# Autodesk Inventor assembly: стенка
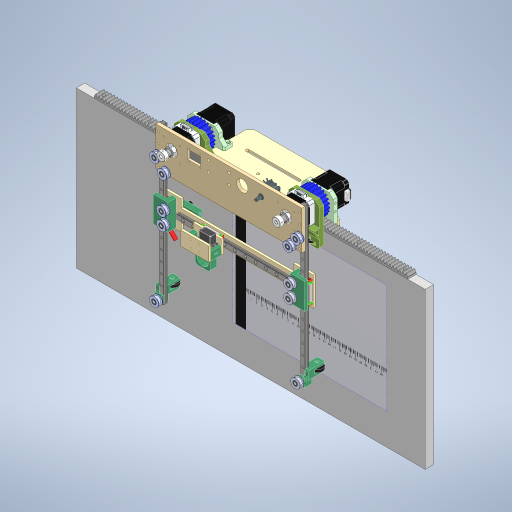
[picture p0: Inventor's stored thumbnail of the model, 512x512]
Saved by Autodesk Inventor 2023.1 (Build 271208000, 208)
## iProperties
Created: 2025-12-01
Part Number: стенка
Document SubType Name: Assembly
Designer: DELL
Author: DELL
## Documents named in this file (9)
- C:\Users\DELL\reposGitHub\VSOSH25-26\models\poligon\poligon.iam
- C:\Users\DELL\reposGitHub\VSOSH25-26\models\plotter\стенка.ipt
- C:\Users\DELL\reposGitHub\VSOSH25-26\models\import\m2_20.ipt
- C:\Users\DELL\reposGitHub\VSOSH25-26\models\actuator\actuator.iam
- C:\Users\DELL\reposGitHub\VSOSH25-26\models\actuator\лист.ipt
- C:\Users\DELL\reposGitHub\VSOSH25-26\models\plotter\plotter_new.iam
- C:\Users\DELL\reposGitHub\VSOSH25-26\models\actuator\actuator_MIR.iam
- C:\Users\DELL\reposGitHub\VSOSH25-26\models\actuator\фанера.ipt
- C:\Users\DELL\reposGitHub\VSOSH25-26\models\ex\фанера_для_электр.ipt
## Components (10 placed, 8 different names)
1. стенка:1 — Совмещение:1, Совмещение:2, Совмещение:4, Совмещение:6, Заподлицо:3, Совмещение:9, Совмещение:10, Совмещение:21
2. m2_20:1 — Совмещение:5, Совмещение:6
3. m2_20:2 — Совмещение:1, Совмещение:2, Совмещение:3
4. m2_20:3 — Совмещение:3, Совмещение:4, Совмещение:5, Заподлицо:1
5. actuator:1 [sub-assembly] — Заподлицо:1, Заподлицо:5, Совмещение:11, Совмещение:14, Совмещение:16, Совмещение:20, Совмещение:21, Совмещение:22
6. лист:1 — Заподлицо:3, Совмещение:9, Совмещение:10
7. plotter_new:1 [sub-assembly] — Заподлицо:5, Совмещение:11, Совмещение:14, Совмещение:15, Совмещение:19
8. actuator_MIR:1 [sub-assembly] — Совмещение:17, Заподлицо:6, Заподлицо:7
9. фанера:1 — Совмещение:16, Совмещение:17, Совмещение:19, Совмещение:20
10. фанера_для_электр:1 — Заподлицо:6, Заподлицо:7, Совмещение:22
## Relationships (22: Mate 17, Flush 5)
- Совмещение:1 [Mate] (33.5 mm): стенка:1 ↔ m2_20:2
- Совмещение:2 [Mate]: стенка:1 ↔ m2_20:2
- Совмещение:3 [Mate]: m2_20:2 ↔ m2_20:3
- Совмещение:4 [Mate]: стенка:1 ↔ m2_20:3
- Совмещение:5 [Mate]: m2_20:1 ↔ m2_20:3
- Совмещение:6 [Mate]: стенка:1 ↔ m2_20:1
- Заподлицо:1 [Flush]: m2_20:3 ↔ actuator:1
- Заподлицо:3 [Flush]: стенка:1 ↔ лист:1
- Совмещение:9 [Mate] (30 mm): стенка:1 ↔ лист:1
- Совмещение:10 [Mate] (300 mm): стенка:1 ↔ лист:1
- Заподлицо:5 [Flush]: actuator:1 ↔ plotter_new:1
- Совмещение:11 [Mate]: actuator:1 ↔ plotter_new:1
- Совмещение:14 [Mate]: actuator:1 ↔ plotter_new:1
- Совмещение:15 [Mate] (-140.4 mm): plotter_new:1
- Совмещение:16 [Mate]: actuator:1 ↔ фанера:1
- Совмещение:17 [Mate]: actuator_MIR:1 ↔ фанера:1
- Совмещение:19 [Mate]: plotter_new:1 ↔ фанера:1
- Совмещение:20 [Mate]: actuator:1 ↔ фанера:1
- Совмещение:21 [Mate] (-28.4 mm): стенка:1 ↔ actuator:1
- Заподлицо:6 [Flush]: actuator_MIR:1 ↔ фанера_для_электр:1
- Заподлицо:7 [Flush]: actuator_MIR:1 ↔ фанера_для_электр:1
- Совмещение:22 [Mate]: actuator:1 ↔ фанера_для_электр:1
